# Autodesk Inventor assembly: Spine
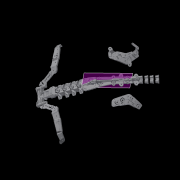
[picture p0: Inventor's stored thumbnail of the model, 180x180]
Saved by Autodesk Inventor 2015 (Build 190159000, 159)
## iProperties
Created: 2015-01-04
Part Number: Spine
Document SubType Name: Assembly
Designer: Val
Mass: 915.202 g
Surface Area: 4175.8 cm^2
Volume: 915.202 cm^3
Density: 1 g/cm^3
Author: Val
## Documents named in this file (15)
- F:\Exo\Models\3D\Spine.iam
- F:\Exo\Models\3D\SpineMiddleRight.ipt
- F:\Exo\Models\3D\SpineBottom.ipt
- F:\Exo\Models\3D\SpineCoverMiddle.ipt
- F:\Exo\Models\3D\SpineMiddleLeft.ipt
- F:\Exo\Models\3D\SpineCoverLeft.ipt
- F:\Exo\Models\3D\SpineCoverRight.ipt
- F:\Exo\Models\3D\SpineMiddleTop.ipt
- F:\Exo\Models\3D\SpineTopMiddleConnector.ipt
- F:\Exo\Models\3D\SpineNeckLinkConnector.ipt
- F:\Exo\Models\3D\SpineTop.ipt
- F:\Exo\Models\3D\Pelvis.iam
- F:\Exo\Models\3D\ShoulderLeft.iam
- F:\Exo\Models\3D\ShoulderRight.ipt
- F:\Exo\Models\3D\NeckLink.ipt
## Components (17 placed, 14 different names)
1. SpineMiddleRight:1 — Mate:12, Mate:17, Mate:23, Flush:2, Mate:30, Mate:38, Flush:5, Flush:6, Angle:4, Flush:7, Mate:48, Mate:53, Mate:54
2. SpineBottom:1 — Mate:12, Mate:17, Mate:21, Mate:37, Angle:1, Flush:3, Flush:4, Mate:41, Angle:6, Angle:7
3. SpineCoverMiddle:1 — Mate:21, Mate:23, Mate:37
4. SpineMiddleLeft:1 — Mate:28, Mate:30, Mate:40, Angle:1, Mate:46, Mate:52
5. SpineCoverLeft:1 — Mate:40, Flush:3, Flush:4, Mate:41
6. SpineCoverRight:1 — Mate:38, Flush:5
7. SpineMiddleTop:1 — Flush:6, Flush:7, Mate:48, Flush:8, Angle:5
8. SpineNeckLinkConnector:1 — Mate:46, Angle:4
9. SpineTopMiddleConnector:2 — Mate:52
10. SpineTop:1 — Flush:8, Angle:5, Flush:9, Mate:58
11. Pelvis:1 [sub-assembly] — Angle:6, Angle:7
12. ShoulderLeft:1 [sub-assembly]
13. ShoulderRight:1
14. SpineTopMiddleConnector:3 — Mate:53, Mate:54
15. NeckLink:1 — Flush:9, Flush:10, Mate:57
16. NeckLink:2 — Flush:10, Mate:56
17. NeckLink:3 — Mate:56, Mate:57, Mate:58
## Relationships (32: Mate 18, Flush 9, Angle 5)
- Mate:12: SpineMiddleRight:1 ↔ SpineBottom:1
- Mate:17: SpineMiddleRight:1 ↔ SpineBottom:1
- Mate:21: SpineBottom:1 ↔ SpineCoverMiddle:1
- Mate:23: SpineMiddleRight:1 ↔ SpineCoverMiddle:1
- Flush:2: SpineMiddleRight:1
- Mate:28: SpineMiddleLeft:1
- Mate:30: SpineMiddleRight:1 ↔ SpineMiddleLeft:1
- Mate:37: SpineBottom:1 ↔ SpineCoverMiddle:1
- Mate:38: SpineMiddleRight:1 ↔ SpineCoverRight:1
- Mate:40: SpineMiddleLeft:1 ↔ SpineCoverLeft:1
- Angle:1: SpineBottom:1 ↔ SpineMiddleLeft:1
- Flush:3: SpineBottom:1 ↔ SpineCoverLeft:1
- Flush:4: SpineBottom:1 ↔ SpineCoverLeft:1
- Mate:41: SpineBottom:1 ↔ SpineCoverLeft:1
- Flush:5: SpineMiddleRight:1 ↔ SpineCoverRight:1
- Flush:6: SpineMiddleRight:1 ↔ SpineMiddleTop:1
- Mate:46: SpineMiddleLeft:1 ↔ SpineNeckLinkConnector:1
- Angle:4: SpineMiddleRight:1 ↔ SpineNeckLinkConnector:1
- Flush:7: SpineMiddleRight:1 ↔ SpineMiddleTop:1
- Mate:48: SpineMiddleRight:1 ↔ SpineMiddleTop:1
- Mate:52: SpineMiddleLeft:1 ↔ SpineTopMiddleConnector:2
- Flush:8: SpineMiddleTop:1 ↔ SpineTop:1
- Angle:5: SpineMiddleTop:1 ↔ SpineTop:1
- Angle:6: SpineBottom:1 ↔ Pelvis:1
- Angle:7: SpineBottom:1 ↔ Pelvis:1
- Mate:53: SpineMiddleRight:1 ↔ SpineTopMiddleConnector:3
- Mate:54: SpineMiddleRight:1 ↔ SpineTopMiddleConnector:3
- Flush:9: SpineTop:1 ↔ NeckLink:1
- Flush:10: NeckLink:1 ↔ NeckLink:2
- Mate:56: NeckLink:2 ↔ NeckLink:3
- Mate:57: NeckLink:1 ↔ NeckLink:3
- Mate:58: SpineTop:1 ↔ NeckLink:3
